# Autodesk Inventor assembly: Mold Design1
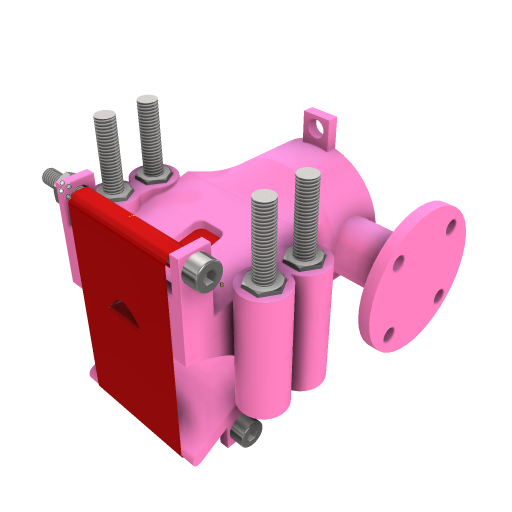
[picture p0: Inventor's stored thumbnail of the model, 512x512]
Saved by Autodesk Inventor 2024 (Build 280153000, 153)
## iProperties
Created: 2023-04-14
Part Number: Mold Design1
Document SubType Name: Assembly
Designer: ferna
Author: ferna
## Documents named in this file (8)
- C:\Users\ferna\OneDrive - Universidad Católica de Chile\Bocas\RobotFlautista\Mold Design1\Mold Design1.iam
- C:\Users\ferna\OneDrive - Universidad Católica de Chile\Bocas\RobotFlautista\nueva_boca_3 - Copy (2).ipt
- C:\Users\ferna\OneDrive - Universidad Católica de Chile\Bocas\RobotFlautista\nueva_boca_3 - Copy (3).ipt
- C:\Users\ferna\OneDrive - Universidad Católica de Chile\Bocas\RobotFlautista\nueva_boca_3 - Copy.ipt
- C:\Users\ferna\OneDrive - Universidad Católica de Chile\Bocas\RobotFlautista\AS 1112 - M5  Type 5.ipt
- C:\Users\ferna\OneDrive - Universidad Católica de Chile\Bocas\RobotFlautista\perno_largo.ipt
- C:\Users\ferna\OneDrive - Universidad Católica de Chile\Bocas\RobotFlautista\ANSI B18.3.1M - M4x0.7 x 50(2).ipt
- C:\Users\ferna\OneDrive - Universidad Católica de Chile\Bocas\RobotFlautista\AS 1112 - M4(2).ipt
## Components (15 placed, 7 different names)
1. nueva_boca_3 - Copy (2):1 — Mate:1, Mate:2, Mate:3, Mate:4, Mate:5, Mate:6
2. nueva_boca_3 - Copy (3):1 — Mate:4, Mate:5, Mate:6, Mate:12, Mate:13, Mate:14, Mate:15, Mate:16, Mate:19, Mate:22, Angle:1, Angle:2, Angle:3, Angle:4, Mate:25
3. nueva_boca_3 - Copy:1 — Mate:1, Mate:2, Mate:3, Mate:17, Mate:20, Mate:21, Mate:23, Mate:24
4. AS 1112 (2) - Metric M5  Type 5:1 — Mate:18, Angle:2, Flush:1
5. AS 1112 (2) - Metric M5  Type 5:2 — Flush:2, Angle:3
6. AS 1112 (2) - Metric M5  Type 5:3 — Mate:22, Angle:1, Flush:1, Flush:2, Flush:3
7. AS 1112 (2) - Metric M5  Type 5:4 — Flush:3, Angle:4
8. perno_largo:1 — Mate:13, Mate:18, Mate:23
9. perno_largo:2 — Mate:12, Flush:4
10. perno_largo:3 — Mate:15, Mate:24, Flush:4
11. perno_largo:4 — Mate:14, Mate:21
12. Broached Socket Head Cap Screw - Metric M4x0.7 x 50:1 — Mate:16, Mate:25, Flush:5
13. AS 1112 (4) - Metric M4:1 — Mate:19
14. Broached Socket Head Cap Screw - Metric M4x0.7 x 50:2 — Mate:17, Flush:5
15. AS 1112 (4) - Metric M4:2 — Mate:20
## Relationships (34: Mate 25, Flush 5, Angle 4)
- Mate:1: nueva_boca_3 - Copy (2):1 ↔ nueva_boca_3 - Copy:1
- Mate:2: nueva_boca_3 - Copy (2):1 ↔ nueva_boca_3 - Copy:1
- Mate:3: nueva_boca_3 - Copy (2):1 ↔ nueva_boca_3 - Copy:1
- Mate:4: nueva_boca_3 - Copy (2):1 ↔ nueva_boca_3 - Copy (3):1
- Mate:5: nueva_boca_3 - Copy (2):1 ↔ nueva_boca_3 - Copy (3):1
- Mate:6: nueva_boca_3 - Copy (2):1 ↔ nueva_boca_3 - Copy (3):1
- [Mate]: AS 1112 (2) - Metric M5  Type 5:3 ↔ perno_largo:4
- [Mate]: AS 1112 (2) - Metric M5  Type 5:2 ↔ perno_largo:2
- [Mate]: AS 1112 (2) - Metric M5  Type 5:4 ↔ perno_largo:3
- [Mate]: Broached Socket Head Cap Screw - Metric M4x0.7 x 50:1 ↔ AS 1112 (4) - Metric M4:1
- [Mate]: Broached Socket Head Cap Screw - Metric M4x0.7 x 50:2 ↔ AS 1112 (4) - Metric M4:2
- Mate:12: nueva_boca_3 - Copy (3):1 ↔ perno_largo:2
- Mate:13: nueva_boca_3 - Copy (3):1 ↔ perno_largo:1
- Mate:14: nueva_boca_3 - Copy (3):1 ↔ perno_largo:4
- Mate:15: nueva_boca_3 - Copy (3):1 ↔ perno_largo:3
- Mate:16: nueva_boca_3 - Copy (3):1 ↔ Broached Socket Head Cap Screw - Metric M4x0.7 x 50:1
- Mate:17: nueva_boca_3 - Copy:1 ↔ Broached Socket Head Cap Screw - Metric M4x0.7 x 50:2
- Mate:18: AS 1112 (2) - Metric M5  Type 5:1 ↔ perno_largo:1
- Mate:19: nueva_boca_3 - Copy (3):1 ↔ AS 1112 (4) - Metric M4:1
- Mate:20: nueva_boca_3 - Copy:1 ↔ AS 1112 (4) - Metric M4:2
- Mate:21: nueva_boca_3 - Copy:1 ↔ perno_largo:4
- Mate:22: nueva_boca_3 - Copy (3):1 ↔ AS 1112 (2) - Metric M5  Type 5:3
- Angle:1 (180 deg): nueva_boca_3 - Copy (3):1 ↔ AS 1112 (2) - Metric M5  Type 5:3
- Angle:2 (0 deg): nueva_boca_3 - Copy (3):1 ↔ AS 1112 (2) - Metric M5  Type 5:1
- Flush:1: AS 1112 (2) - Metric M5  Type 5:1 ↔ AS 1112 (2) - Metric M5  Type 5:3
- Mate:23: nueva_boca_3 - Copy:1 ↔ perno_largo:1
- Flush:2: AS 1112 (2) - Metric M5  Type 5:2 ↔ AS 1112 (2) - Metric M5  Type 5:3
- Flush:3: AS 1112 (2) - Metric M5  Type 5:3 ↔ AS 1112 (2) - Metric M5  Type 5:4
- Angle:3 (0 deg): nueva_boca_3 - Copy (3):1 ↔ AS 1112 (2) - Metric M5  Type 5:2
- Angle:4 (0 deg): nueva_boca_3 - Copy (3):1 ↔ AS 1112 (2) - Metric M5  Type 5:4
- Mate:24: nueva_boca_3 - Copy:1 ↔ perno_largo:3
- Flush:4: perno_largo:2 ↔ perno_largo:3
- Mate:25: nueva_boca_3 - Copy (3):1 ↔ Broached Socket Head Cap Screw - Metric M4x0.7 x 50:1
- Flush:5: Broached Socket Head Cap Screw - Metric M4x0.7 x 50:1 ↔ Broached Socket Head Cap Screw - Metric M4x0.7 x 50:2
